# Autodesk Inventor assembly: Molde_Full
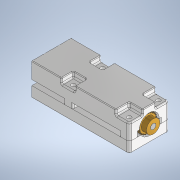
[picture p0: Inventor's stored thumbnail of the model, 180x180]
Saved by Autodesk Inventor 2020.2 (Build 242310000, 310)
## iProperties
Created: 2020-12-05
Part Number: Molde_Full
Document SubType Name: Assembly
Designer: Acer
Author: Acer
## Documents named in this file (6)
- C:\Users\Acer\Desktop\2020 LARC\2020_LARC\first_floor\Dribbler\Molde_Full.iam
- C:\Users\Acer\Desktop\2020 LARC\2020_LARC\first_floor\Dribbler\MoldeA.ipt
- C:\Users\Acer\Desktop\2020 LARC\2020_LARC\first_floor\Dribbler\MoldeB.ipt
- C:\Users\Acer\Desktop\2020 LARC\2020_LARC\first_floor\Dribbler\Eixo.ipt
- C:\Users\Acer\Desktop\2020 LARC\2020_LARC\first_floor\Dribbler\Kugellager 685-ZZ-C3.ipt
- C:\Users\Acer\Desktop\2020 LARC\2020_LARC\first_floor\Dribbler\Ritzel schmal z26_machined.ipt
## Components (6 placed, 4 different names)
1. Dribblerschnecke:1 — Flush:1, Flush:2, Mate:1, Mate:2, Mate:3
2. Dribblerschnecke:2 — Flush:1, Flush:2, Mate:1
3. Eixo:1 — Mate:2, Mate:3, Mate:4, Mate:5, Mate:6, Mate:7, Mate:8
4. Kugellager 685-ZZ-C3:1 — Mate:4, Mate:7, Mate:9
5. Kugellager 685-ZZ-C3:2 — Mate:5, Mate:6
6. Ritzel schmal z=26:1 — Mate:8, Mate:9
## Relationships (11: Mate 9, Flush 2)
- Flush:1: Dribblerschnecke:1 ↔ Dribblerschnecke:2
- Flush:2: Dribblerschnecke:1 ↔ Dribblerschnecke:2
- Mate:1: Dribblerschnecke:1 ↔ Dribblerschnecke:2
- Mate:2: Dribblerschnecke:1 ↔ Eixo:1
- Mate:3 (-2 mm): Dribblerschnecke:1 ↔ Eixo:1
- Mate:4: Eixo:1 ↔ Kugellager 685-ZZ-C3:1
- Mate:5: Eixo:1 ↔ Kugellager 685-ZZ-C3:2
- Mate:6: Eixo:1 ↔ Kugellager 685-ZZ-C3:2
- Mate:7: Eixo:1 ↔ Kugellager 685-ZZ-C3:1
- Mate:8: Eixo:1 ↔ Ritzel schmal z=26:1
- Mate:9: Kugellager 685-ZZ-C3:1 ↔ Ritzel schmal z=26:1
